# Autodesk Inventor assembly: Power 220 AC Cable
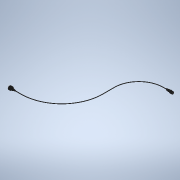
[picture p0: Inventor's stored thumbnail of the model, 180x180]
Saved by Autodesk Inventor 2020 (Build 240168000, 168)
## iProperties
Created: 2020-07-06
Part Number: Power 220 AC Cable
Document SubType Name: Assembly
Designer: Bruno
Author: Bruno
## Documents named in this file (4)
- C:\Users\Juan\Desktop\CAD Inventor\Power 220 AC Cable.iam
- C:\Users\Juan\Desktop\CAD Inventor\IEC 320 C13 Cable End.ipt
- C:\Users\Juan\Desktop\CAD Inventor\Cable 220V - 2.5in - 1.5m.ipt
- C:\Users\Juan\Desktop\CAD Inventor\AC plug.ipt
## Components (3 placed, 3 different names)
1. IEC 320 C13 Cable End:1 — Flush:1, Flush:3
2. Cable 220V - 2.5in - 1.5m:1 — Flush:1, Flush:3, Cylindrical:1
3. AC plug:1 — Cylindrical:1
## Relationships (3: Flush 2, CylindricalJoint 1)
- Flush:1: IEC 320 C13 Cable End:1 ↔ Cable 220V - 2.5in - 1.5m:1
- Flush:3: IEC 320 C13 Cable End:1 ↔ Cable 220V - 2.5in - 1.5m:1
- Cylindrical:1: Cable 220V - 2.5in - 1.5m:1 ↔ AC plug:1
